# Autodesk Inventor assembly: powerbank
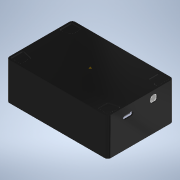
[picture p0: Inventor's stored thumbnail of the model, 180x180]
Saved by Autodesk Inventor 2021 (Build 250183000, 183)
## iProperties
Created: 2020-12-16
Part Number: powerbank
Document SubType Name: Assembly
Designer: oskar
Author: oskar
## Documents named in this file (3)
- C:\Users\oskar\Dropbox\Dokument\Projekt\Powerbank-MDP-XP\cad\powerbank.iam
- C:\Users\oskar\Dropbox\Dokument\Projekt\Powerbank-MDP-XP\cad\pcb_complete.iam
- C:\Users\oskar\Dropbox\Dokument\Projekt\Powerbank-MDP-XP\cad\enclosure_bot.ipt
## Components (2 placed, 2 different names)
1. pcb_complete:1 [sub-assembly] — Flush:1, Flush:2
2. enclosure_bot:1 — Flush:1, Flush:2
## Relationships (2: Flush 2)
- Flush:1: pcb_complete:1 ↔ enclosure_bot:1
- Flush:2 (5 mm): pcb_complete:1 ↔ enclosure_bot:1
